# Autodesk Inventor assembly: Non Pass Through EndCap
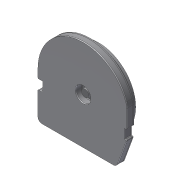
[picture p0: Inventor's stored thumbnail of the model, 180x180]
Saved by Autodesk Inventor 2015 (Build 190159000, 159)
## iProperties
Created: 2015-07-21
Part Number: Non Pass Through EndCap
Document SubType Name: Assembly
Designer: JR
Author: JR
## Documents named in this file (7)
- F:\OpenROV\2.8\Electronics Tube\EndCaps\Non Pass Through\Non Pass Through EndCap.iam
- F:\OpenROV\2.8\Electronics Tube\EndCaps\Non Pass Through\NPT Outer Gland.ipt
- F:\OpenROV\2.8\Electronics Tube\EndCaps\Non Pass Through\NPT Inside Gland.ipt
- F:\OpenROV\2.8\Electronics Tube\EndCaps\Non Pass Through\NPT Gland.ipt
- F:\OpenROV\2.8\Electronics Tube\EndCaps\Non Pass Through\NPT Flange Outer.ipt
- F:\OpenROV\2.8\Electronics Tube\EndCaps\Non Pass Through\NPT Flange Inner.ipt
- F:\OpenROV\Syringe.ipt
## Components (7 placed, 6 different names)
1. NPT Outer Gland:1 — Mate:1, Mate:2, Mate:5, Mate:6
2. NPT Inside Gland:1 — Mate:3, Mate:4, Flush:3, Mate:11
3. NPT Gland:1 — Mate:1, Mate:2, Mate:3, Mate:4
4. NPT Flange Outer:1 — Mate:9, Mate:10, Flush:2
5. NPT Flange Inner:1 — Mate:7, Mate:8, Flush:1, Mate:9, Mate:10, Flush:2
6. NPT Flange Outer:2 — Mate:5, Mate:6, Mate:7, Mate:8, Flush:1
7. Syringe:1 — Flush:3, Mate:11
## Relationships (14: Mate 11, Flush 3)
- Mate:1: NPT Outer Gland:1 ↔ NPT Gland:1
- Mate:2: NPT Outer Gland:1 ↔ NPT Gland:1
- Mate:3: NPT Inside Gland:1 ↔ NPT Gland:1
- Mate:4: NPT Inside Gland:1 ↔ NPT Gland:1
- Mate:5: NPT Outer Gland:1 ↔ NPT Flange Outer:2
- Mate:6: NPT Outer Gland:1 ↔ NPT Flange Outer:2
- Mate:7: NPT Flange Inner:1 ↔ NPT Flange Outer:2
- Mate:8: NPT Flange Inner:1 ↔ NPT Flange Outer:2
- Flush:1: NPT Flange Inner:1 ↔ NPT Flange Outer:2
- Mate:9: NPT Flange Outer:1 ↔ NPT Flange Inner:1
- Mate:10: NPT Flange Outer:1 ↔ NPT Flange Inner:1
- Flush:2: NPT Flange Outer:1 ↔ NPT Flange Inner:1
- Flush:3: NPT Inside Gland:1 ↔ Syringe:1
- Mate:11: NPT Inside Gland:1 ↔ Syringe:1
